# Autodesk Inventor assembly: SUP_000_FullSuperstructure
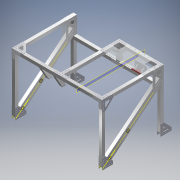
[picture p0: Inventor's stored thumbnail of the model, 180x180]
Saved by Autodesk Inventor 2018.3 (Build 223284000, 284)
## iProperties
Created: 2020-01-26
Part Number: SUP_000_FullSuperstructure
Document SubType Name: Assembly
Designer: user
Mass: 1586.6 g
Surface Area: 7435.44 cm^2
Volume: 587.63 cm^3
Density: 2.7 g/cm^3
Author: user
## Documents named in this file (21)
- C:\Users\22barlalex\Documents\GrabCAD\Infinite Recharge 2020\Build season\SUP_000_FullSuperstructure.iam
- C:\Users\22barlalex\Documents\GrabCAD\Infinite Recharge 2020\Build season\SUP_001_CornerVertical.ipt
- C:\Users\22barlalex\Documents\GrabCAD\Infinite Recharge 2020\Build season\SUP_004_TopConnectorBar.ipt
- C:\Users\22barlalex\Documents\GrabCAD\Infinite Recharge 2020\Build season\SUP_005_Middle ConnectorBar.ipt
- C:\Users\22barlalex\Documents\GrabCAD\Infinite Recharge 2020\Build season\SUP_007_ConnectorBar.ipt
- C:\Users\22barlalex\Documents\GrabCAD\Infinite Recharge 2020\Build season\SUP_008_FrontCornerVertical.ipt
- C:\Users\22barlalex\Documents\GrabCAD\Infinite Recharge 2020\Build season\SUP_003_TGusset.ipt
- C:\Users\22barlalex\Documents\GrabCAD\Infinite Recharge 2020\Build season\SUP_002_90DegreeGusset.ipt
- C:\Users\22barlalex\Documents\GrabCAD\Infinite Recharge 2020\Build season\SUP_009_90DegreeGussetCorner.ipt
- C:\Users\22barlalex\Documents\GrabCAD\Infinite Recharge 2020\Build season\SUP_010_4BarBar.ipt
- C:\Users\22barlalex\Documents\GrabCAD\Infinite Recharge 2020\Build season\DGB STEP\217-2731_0_500_flanged_bearing.ipt
- C:\Users\22barlalex\Documents\GrabCAD\Infinite Recharge 2020\Build season\SUP_013_NewerTop4BarBarGusset.ipt
- C:\Users\22barlalex\Documents\GrabCAD\Infinite Recharge 2020\Build season\SUP_014_HALFMiddleConnectorBar.ipt
- C:\Users\22barlalex\Documents\GrabCAD\Infinite Recharge 2020\Build season\SUP_015_ShortCenterToptoBottomSupport.ipt
- C:\Users\22barlalex\Documents\GrabCAD\Infinite Recharge 2020\Build season\SUP_016_SmallerTGusset.ipt
- C:\Users\22barlalex\Documents\GrabCAD\Infinite Recharge 2020\Build season\SUP_017_CutNewerTop4BarBarGusset.ipt
- C:\Users\22barlalex\Documents\GrabCAD\Infinite Recharge 2020\Build season\SUP_018_120Gusset.ipt
- C:\Users\22barlalex\Documents\GrabCAD\Infinite Recharge 2020\Build season\Electronics\LimelightCaseAssembly.iam
- C:\Users\22barlalex\Documents\GrabCAD\Infinite Recharge 2020\Build season\SUP_021_LexanShield.ipt
- C:\Users\22barlalex\Documents\GrabCAD\Infinite Recharge 2020\Build season\SUP_022_NEWClimberSupport.ipt
- C:\Users\22barlalex\Documents\GrabCAD\Infinite Recharge 2020\Build season\SUP_012_Bottom4BarBarGusset.ipt
## Components (54 placed, 20 different names)
1. SUP_001_CornerVertical:1 — Flush:1, Flush:2, Mate:6, Flush:9, Flush:16, Mate:19, Mate:51, Flush:70, Flush:74, Mate:66, Flush:95, Mate:69, Flush:101, Flush:114, Flush:115, Mate:89, Mate:91, Flush:121
2. SUP_001_CornerVertical:2 — Flush:1, Flush:2, Mate:4, Flush:7, Flush:33, Mate:29, Mate:53, Flush:71, Mate:55, Flush:75, Mate:56, Mate:65, Flush:93, Mate:70, Flush:102, Mate:74, Flush:116, Flush:117, Mate:88, Flush:118, Mate:90
3. SUP_004_TopConnectorBar:1 — Mate:4, Flush:7, Flush:8, Mate:15, Flush:17, Mate:16, Flush:29, Mate:27, Mate:41, Flush:50, Flush:51, Mate:42, Flush:77, Flush:112
4. SUP_004_TopConnectorBar:2 — Flush:8, Mate:6, Flush:9, Mate:12, Flush:16, Mate:14, Mate:17, Flush:18, Mate:18, Mate:19, Flush:22, Mate:23, Flush:37, Mate:34, Mate:54, Flush:73, Flush:100
5. SUP_005_Middle ConnectorBar:2 — Mate:12, Mate:14, Flush:24, Mate:24, Mate:25, Flush:25, Flush:38, Flush:45, Flush:49, Mate:45, Flush:58, Mate:57, Flush:78, Mate:82, Mate:85, Mate:96, Mate:97
6. SUP_008_FrontCornerVertical:1 — Mate:15, Flush:17, Mate:16, Flush:28, Mate:43, Flush:53, Flush:54, Flush:57, Flush:122, Mate:92, Mate:93, Flush:123, Flush:129
7. SUP_008_FrontCornerVertical:2 — Mate:17, Flush:18, Mate:18, Flush:21, Flush:23, Mate:44, Flush:55, Flush:56, Mate:99, Mate:100
8. SUP_003_TGusset:2 — Mate:25, Flush:25
9. SUP_002_90DegreeGusset:2 — Flush:21, Flush:22, Mate:23
10. SUP_009_90DegreeGussetCorner:5 — Flush:23, Flush:24, Mate:24
11. SUP_002_90DegreeGusset:16 — Flush:33, Mate:29
12. SUP_002_90DegreeGusset:6 — Flush:28, Flush:29, Mate:27
13. SUP_002_90DegreeGusset:9 — Flush:37, Flush:38, Mate:34
14. SUP_003_TGusset:3 — Flush:45
15. SUP_009_90DegreeGussetCorner:1 — Mate:41, Flush:49, Flush:50
16. SUP_009_90DegreeGussetCorner:2 — Flush:51, Mate:42
17. SUP_010_4BarBar:1 — Mate:43, Flush:53, Flush:54, Insert:1, Insert:2, Insert:7, Insert:8
18. SUP_010_4BarBar:2 — Mate:44, Flush:55, Flush:56, Insert:3, Insert:4, Insert:5, Insert:6
19. SUP_009_90DegreeGussetCorner:3 — Mate:45, Flush:57, Flush:58
20. SUP_005_Middle ConnectorBar:3 — Mate:51, Flush:70, Mate:56, Mate:59, Flush:80, Mate:64, Flush:91, Flush:92, Flush:94, Mate:68, Flush:105, Mate:73
21. 217-2731_0_500_flanged_bearing:1 — Insert:3
22. 217-2731_0_500_flanged_bearing:2 — Insert:2
23. 217-2731_0_500_flanged_bearing:3 — Insert:8
24. 217-2731_0_500_flanged_bearing:4 — Insert:7
25. 217-2731_0_500_flanged_bearing:5 — Insert:6
26. 217-2731_0_500_flanged_bearing:6 — Insert:5
27. 217-2731_0_500_flanged_bearing:7 — Insert:4
28. 217-2731_0_500_flanged_bearing:8 — Insert:1
29. SUP_013_NewerTop4BarBarGusset:1 — Mate:53, Flush:71
30. SUP_013_NewerTop4BarBarGusset:2 — Mate:54, Flush:73, Flush:74
31. SUP_014_HALFMiddleConnectorBar:1 — Mate:55, Flush:75, Flush:77, Mate:58, Flush:79, Mate:60, Mate:61, Flush:83, Flush:86, Flush:87, Flush:104, Mate:72, Flush:111
32. SUP_007_ConnectorBar:1 — Mate:57, Flush:78, Mate:58, Flush:79, Flush:81, Mate:62, Flush:103, Mate:79, Mate:98
33. SUP_015_ShortCenterToptoBottomSupport:1 — Mate:59, Flush:80, Flush:81, Mate:60, Flush:82, Flush:90, Flush:98
34. SUP_002_90DegreeGusset:10 — Flush:86, Mate:62, Flush:87
35. SUP_002_90DegreeGusset:11 — Mate:61, Flush:82, Flush:83
36. SUP_003_TGusset:5 — Mate:64, Flush:90, Flush:91, Flush:99
37. SUP_003_TGusset:6 — Mate:66, Flush:94, Flush:95
38. SUP_003_TGusset:7 — Mate:65, Flush:92, Flush:93
39. SUP_016_SmallerTGusset:1 — Mate:68, Flush:98, Flush:99
40. SUP_017_CutNewerTop4BarBarGusset:1 — Mate:69, Flush:100, Flush:101
41. SUP_018_120Gusset:1 — Mate:70, Flush:102
42. SUP_009_90DegreeGussetCorner:4 — Flush:103, Flush:104, Mate:72
43. LimelightCaseAssembly:1 [sub-assembly] — Flush:105, Mate:73, Mate:74
44. SUP_021_LexanShield:1 — Mate:79, Flush:111, Flush:112
45. SUP_022_NEWClimberSupport:3 — Mate:82, Mate:85, Flush:130
46. SUP_022_NEWClimberSupport:4 — Mate:96, Mate:97, Flush:130, Mate:98
47. SUP_002_90DegreeGusset:12 — Flush:114, Flush:115, Mate:89, Flush:120
48. SUP_002_90DegreeGusset:13 — Flush:116, Flush:117, Mate:88, Flush:119
49. SUP_002_90DegreeGusset:14 — Flush:118, Flush:119, Mate:90
50. SUP_002_90DegreeGusset:15 — Flush:120, Mate:91, Flush:121
51. SUP_012_Bottom4BarBarGusset:1 — Flush:122, Mate:92, Flush:126, Flush:129
52. SUP_012_Bottom4BarBarGusset:2 — Mate:93, Flush:123, Flush:126, Flush:131, Flush:132
53. SUP_012_Bottom4BarBarGusset:3 — Flush:133, Flush:134, Mate:100
54. SUP_012_Bottom4BarBarGusset:4 — Mate:99, Flush:131, Flush:132, Flush:133, Flush:134
## Relationships (137: Flush 75, Mate 54, Insert 8)
- Flush:1: SUP_001_CornerVertical:1 ↔ SUP_001_CornerVertical:2
- Flush:2: SUP_001_CornerVertical:1 ↔ SUP_001_CornerVertical:2
- Mate:4: SUP_001_CornerVertical:2 ↔ SUP_004_TopConnectorBar:1
- Flush:7: SUP_001_CornerVertical:2 ↔ SUP_004_TopConnectorBar:1
- Flush:8: SUP_004_TopConnectorBar:1 ↔ SUP_004_TopConnectorBar:2
- Mate:6: SUP_001_CornerVertical:1 ↔ SUP_004_TopConnectorBar:2
- Flush:9: SUP_001_CornerVertical:1 ↔ SUP_004_TopConnectorBar:2
- Mate:12: SUP_004_TopConnectorBar:2 ↔ SUP_005_Middle ConnectorBar:2
- Flush:16: SUP_001_CornerVertical:1 ↔ SUP_004_TopConnectorBar:2
- Mate:14: SUP_004_TopConnectorBar:2 ↔ SUP_005_Middle ConnectorBar:2
- Mate:15: SUP_004_TopConnectorBar:1 ↔ SUP_008_FrontCornerVertical:1
- Flush:17: SUP_004_TopConnectorBar:1 ↔ SUP_008_FrontCornerVertical:1
- Mate:16: SUP_004_TopConnectorBar:1 ↔ SUP_008_FrontCornerVertical:1
- Mate:17: SUP_004_TopConnectorBar:2 ↔ SUP_008_FrontCornerVertical:2
- Flush:18: SUP_004_TopConnectorBar:2 ↔ SUP_008_FrontCornerVertical:2
- Mate:18: SUP_004_TopConnectorBar:2 ↔ SUP_008_FrontCornerVertical:2
- Mate:19: SUP_001_CornerVertical:1 ↔ SUP_004_TopConnectorBar:2
- Flush:21: SUP_008_FrontCornerVertical:2 ↔ SUP_002_90DegreeGusset:2
- Flush:22: SUP_004_TopConnectorBar:2 ↔ SUP_002_90DegreeGusset:2
- Mate:23: SUP_004_TopConnectorBar:2 ↔ SUP_002_90DegreeGusset:2
- Flush:23: SUP_008_FrontCornerVertical:2 ↔ SUP_009_90DegreeGussetCorner:5
- Flush:24: SUP_005_Middle ConnectorBar:2 ↔ SUP_009_90DegreeGussetCorner:5
- Mate:24: SUP_005_Middle ConnectorBar:2 ↔ SUP_009_90DegreeGussetCorner:5
- Mate:25: SUP_005_Middle ConnectorBar:2 ↔ SUP_003_TGusset:2
- Flush:25: SUP_005_Middle ConnectorBar:2 ↔ SUP_003_TGusset:2
- Flush:28: SUP_008_FrontCornerVertical:1 ↔ SUP_002_90DegreeGusset:6
- Flush:29: SUP_004_TopConnectorBar:1 ↔ SUP_002_90DegreeGusset:6
- Mate:27: SUP_004_TopConnectorBar:1 ↔ SUP_002_90DegreeGusset:6
- Flush:33: SUP_001_CornerVertical:2 ↔ SUP_002_90DegreeGusset:16
- Mate:29: SUP_001_CornerVertical:2 ↔ SUP_002_90DegreeGusset:16
- Flush:37: SUP_004_TopConnectorBar:2 ↔ SUP_002_90DegreeGusset:9
- Flush:38: SUP_005_Middle ConnectorBar:2 ↔ SUP_002_90DegreeGusset:9
- Mate:34: SUP_004_TopConnectorBar:2 ↔ SUP_002_90DegreeGusset:9
- Flush:45: SUP_005_Middle ConnectorBar:2 ↔ SUP_003_TGusset:3
- Mate:41: SUP_004_TopConnectorBar:1 ↔ SUP_009_90DegreeGussetCorner:1
- Flush:49: SUP_005_Middle ConnectorBar:2 ↔ SUP_009_90DegreeGussetCorner:1
- Flush:50: SUP_004_TopConnectorBar:1 ↔ SUP_009_90DegreeGussetCorner:1
- Flush:51: SUP_004_TopConnectorBar:1 ↔ SUP_009_90DegreeGussetCorner:2
- Mate:42: SUP_004_TopConnectorBar:1 ↔ SUP_009_90DegreeGussetCorner:2
- Mate:43: SUP_008_FrontCornerVertical:1 ↔ SUP_010_4BarBar:1
- Flush:53: SUP_008_FrontCornerVertical:1 ↔ SUP_010_4BarBar:1
- Flush:54: SUP_008_FrontCornerVertical:1 ↔ SUP_010_4BarBar:1
- Mate:44: SUP_008_FrontCornerVertical:2 ↔ SUP_010_4BarBar:2
- Flush:55: SUP_008_FrontCornerVertical:2 ↔ SUP_010_4BarBar:2
- Flush:56: SUP_008_FrontCornerVertical:2 ↔ SUP_010_4BarBar:2
- Mate:45: SUP_005_Middle ConnectorBar:2 ↔ SUP_009_90DegreeGussetCorner:3
- Flush:57: SUP_008_FrontCornerVertical:1 ↔ SUP_009_90DegreeGussetCorner:3
- Flush:58: SUP_005_Middle ConnectorBar:2 ↔ SUP_009_90DegreeGussetCorner:3
- Mate:51: SUP_001_CornerVertical:1 ↔ SUP_005_Middle ConnectorBar:3
- Flush:70: SUP_001_CornerVertical:1 ↔ SUP_005_Middle ConnectorBar:3
- Insert:1: SUP_010_4BarBar:1 ↔ 217-2731_0_500_flanged_bearing:8
- Insert:2: SUP_010_4BarBar:1 ↔ 217-2731_0_500_flanged_bearing:2
- Insert:3: SUP_010_4BarBar:2 ↔ 217-2731_0_500_flanged_bearing:1
- Insert:4: SUP_010_4BarBar:2 ↔ 217-2731_0_500_flanged_bearing:7
- Insert:5: SUP_010_4BarBar:2 ↔ 217-2731_0_500_flanged_bearing:6
- Insert:6: SUP_010_4BarBar:2 ↔ 217-2731_0_500_flanged_bearing:5
- Insert:7: SUP_010_4BarBar:1 ↔ 217-2731_0_500_flanged_bearing:4
- Insert:8: SUP_010_4BarBar:1 ↔ 217-2731_0_500_flanged_bearing:3
- Mate:53: SUP_001_CornerVertical:2 ↔ SUP_013_NewerTop4BarBarGusset:1
- Flush:71: SUP_001_CornerVertical:2 ↔ SUP_013_NewerTop4BarBarGusset:1
- Mate:54: SUP_004_TopConnectorBar:2 ↔ SUP_013_NewerTop4BarBarGusset:2
- Flush:73: SUP_004_TopConnectorBar:2 ↔ SUP_013_NewerTop4BarBarGusset:2
- Flush:74: SUP_001_CornerVertical:1 ↔ SUP_013_NewerTop4BarBarGusset:2
- Mate:55: SUP_001_CornerVertical:2 ↔ SUP_014_HALFMiddleConnectorBar:1
- Flush:75: SUP_001_CornerVertical:2 ↔ SUP_014_HALFMiddleConnectorBar:1
- Mate:56: SUP_001_CornerVertical:2 ↔ SUP_005_Middle ConnectorBar:3
- Flush:77: SUP_004_TopConnectorBar:1 ↔ SUP_014_HALFMiddleConnectorBar:1
- Mate:57: SUP_005_Middle ConnectorBar:2 ↔ SUP_007_ConnectorBar:1
- Flush:78: SUP_005_Middle ConnectorBar:2 ↔ SUP_007_ConnectorBar:1
- Mate:58: SUP_014_HALFMiddleConnectorBar:1 ↔ SUP_007_ConnectorBar:1
- Flush:79: SUP_014_HALFMiddleConnectorBar:1 ↔ SUP_007_ConnectorBar:1
- Mate:59: SUP_005_Middle ConnectorBar:3 ↔ SUP_015_ShortCenterToptoBottomSupport:1
- Flush:80: SUP_005_Middle ConnectorBar:3 ↔ SUP_015_ShortCenterToptoBottomSupport:1
- Flush:81: SUP_007_ConnectorBar:1 ↔ SUP_015_ShortCenterToptoBottomSupport:1
- Mate:60: SUP_014_HALFMiddleConnectorBar:1 ↔ SUP_015_ShortCenterToptoBottomSupport:1
- Mate:61: SUP_014_HALFMiddleConnectorBar:1 ↔ SUP_002_90DegreeGusset:11
- Flush:82: SUP_015_ShortCenterToptoBottomSupport:1 ↔ SUP_002_90DegreeGusset:11
- Flush:83: SUP_014_HALFMiddleConnectorBar:1 ↔ SUP_002_90DegreeGusset:11
- Flush:86: SUP_014_HALFMiddleConnectorBar:1 ↔ SUP_002_90DegreeGusset:10
- Mate:62: SUP_007_ConnectorBar:1 ↔ SUP_002_90DegreeGusset:10
- Flush:87: SUP_014_HALFMiddleConnectorBar:1 ↔ SUP_002_90DegreeGusset:10
- Mate:64: SUP_005_Middle ConnectorBar:3 ↔ SUP_003_TGusset:5
- Flush:90: SUP_015_ShortCenterToptoBottomSupport:1 ↔ SUP_003_TGusset:5
- Flush:91: SUP_005_Middle ConnectorBar:3 ↔ SUP_003_TGusset:5
- Mate:65: SUP_001_CornerVertical:2 ↔ SUP_003_TGusset:7
- Flush:92: SUP_005_Middle ConnectorBar:3 ↔ SUP_003_TGusset:7
- Flush:93: SUP_001_CornerVertical:2 ↔ SUP_003_TGusset:7
- Mate:66: SUP_001_CornerVertical:1 ↔ SUP_003_TGusset:6
- Flush:94: SUP_005_Middle ConnectorBar:3 ↔ SUP_003_TGusset:6
- Flush:95: SUP_001_CornerVertical:1 ↔ SUP_003_TGusset:6
- Mate:68: SUP_005_Middle ConnectorBar:3 ↔ SUP_016_SmallerTGusset:1
- Flush:98: SUP_015_ShortCenterToptoBottomSupport:1 ↔ SUP_016_SmallerTGusset:1
- Flush:99: SUP_003_TGusset:5 ↔ SUP_016_SmallerTGusset:1
- Mate:69: SUP_001_CornerVertical:1 ↔ SUP_017_CutNewerTop4BarBarGusset:1
- Flush:100: SUP_004_TopConnectorBar:2 ↔ SUP_017_CutNewerTop4BarBarGusset:1
- Flush:101: SUP_001_CornerVertical:1 ↔ SUP_017_CutNewerTop4BarBarGusset:1
- Mate:70: SUP_001_CornerVertical:2 ↔ SUP_018_120Gusset:1
- Flush:102: SUP_001_CornerVertical:2 ↔ SUP_018_120Gusset:1
- Flush:103: SUP_007_ConnectorBar:1 ↔ SUP_009_90DegreeGussetCorner:4
- Flush:104: SUP_014_HALFMiddleConnectorBar:1 ↔ SUP_009_90DegreeGussetCorner:4
- Mate:72: SUP_014_HALFMiddleConnectorBar:1 ↔ SUP_009_90DegreeGussetCorner:4
- Flush:105: SUP_005_Middle ConnectorBar:3 ↔ LimelightCaseAssembly:1
- Mate:73: SUP_005_Middle ConnectorBar:3 ↔ LimelightCaseAssembly:1
- Mate:74 (106.5276 mm): SUP_001_CornerVertical:2 ↔ LimelightCaseAssembly:1
- Mate:79: SUP_007_ConnectorBar:1 ↔ SUP_021_LexanShield:1
- Flush:111: SUP_014_HALFMiddleConnectorBar:1 ↔ SUP_021_LexanShield:1
- Flush:112: SUP_004_TopConnectorBar:1 ↔ SUP_021_LexanShield:1
- Mate:82: SUP_005_Middle ConnectorBar:2 ↔ SUP_022_NEWClimberSupport:3
- Mate:85: SUP_005_Middle ConnectorBar:2 ↔ SUP_022_NEWClimberSupport:3
- Flush:114: SUP_001_CornerVertical:1 ↔ SUP_002_90DegreeGusset:12
- Flush:115 (-25.4 mm): SUP_001_CornerVertical:1 ↔ SUP_002_90DegreeGusset:12
- Flush:116 (-25.4 mm): SUP_001_CornerVertical:2 ↔ SUP_002_90DegreeGusset:13
- Flush:117: SUP_001_CornerVertical:2 ↔ SUP_002_90DegreeGusset:13
- Mate:88: SUP_001_CornerVertical:2 ↔ SUP_002_90DegreeGusset:13
- Mate:89: SUP_001_CornerVertical:1 ↔ SUP_002_90DegreeGusset:12
- Flush:118: SUP_001_CornerVertical:2 ↔ SUP_002_90DegreeGusset:14
- Flush:119: SUP_002_90DegreeGusset:13 ↔ SUP_002_90DegreeGusset:14
- Mate:90: SUP_001_CornerVertical:2 ↔ SUP_002_90DegreeGusset:14
- Flush:120: SUP_002_90DegreeGusset:12 ↔ SUP_002_90DegreeGusset:15
- Mate:91: SUP_001_CornerVertical:1 ↔ SUP_002_90DegreeGusset:15
- Flush:121: SUP_001_CornerVertical:1 ↔ SUP_002_90DegreeGusset:15
- Flush:122: SUP_008_FrontCornerVertical:1 ↔ SUP_012_Bottom4BarBarGusset:1
- Mate:92: SUP_008_FrontCornerVertical:1 ↔ SUP_012_Bottom4BarBarGusset:1
- Mate:93: SUP_008_FrontCornerVertical:1 ↔ SUP_012_Bottom4BarBarGusset:2
- Flush:123: SUP_008_FrontCornerVertical:1 ↔ SUP_012_Bottom4BarBarGusset:2
- Flush:126: SUP_012_Bottom4BarBarGusset:1 ↔ SUP_012_Bottom4BarBarGusset:2
- Flush:129 (25.4 mm): SUP_008_FrontCornerVertical:1 ↔ SUP_012_Bottom4BarBarGusset:1
- Mate:96: SUP_005_Middle ConnectorBar:2 ↔ SUP_022_NEWClimberSupport:4
- Mate:97: SUP_005_Middle ConnectorBar:2 ↔ SUP_022_NEWClimberSupport:4
- Flush:130 (111.125 mm): SUP_022_NEWClimberSupport:3 ↔ SUP_022_NEWClimberSupport:4
- Mate:98 (19.05 mm): SUP_007_ConnectorBar:1 ↔ SUP_022_NEWClimberSupport:4
- Mate:99: SUP_008_FrontCornerVertical:2 ↔ SUP_012_Bottom4BarBarGusset:4
- Flush:131: SUP_012_Bottom4BarBarGusset:2 ↔ SUP_012_Bottom4BarBarGusset:4
- Flush:132: SUP_012_Bottom4BarBarGusset:2 ↔ SUP_012_Bottom4BarBarGusset:4
- Flush:133: SUP_012_Bottom4BarBarGusset:3 ↔ SUP_012_Bottom4BarBarGusset:4
- Flush:134: SUP_012_Bottom4BarBarGusset:3 ↔ SUP_012_Bottom4BarBarGusset:4
- Mate:100: SUP_008_FrontCornerVertical:2 ↔ SUP_012_Bottom4BarBarGusset:3
